# Autodesk Inventor assembly: raspi
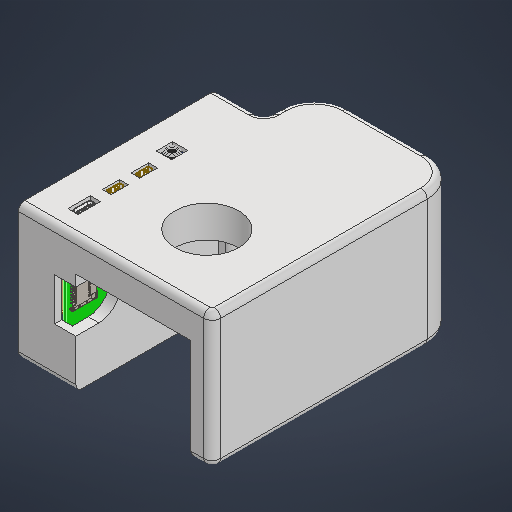
[picture p0: Inventor's stored thumbnail of the model, 512x512]
Saved by Autodesk Inventor 2025.3 (Build 293356030, 356C)
## iProperties
Created: 2025-09-19
Part Number: raspi
Document SubType Name: Assembly
Designer: river
Author: river
## Documents named in this file (4)
- C:\Users\river\OneDrive\Documentos\protesis V2\raspi.iam
- C:\Users\river\OneDrive\Documentos\sync\Part4.ipt
- C:\Users\river\Downloads\self-locking-button-switch-lay37-pbcy-green-1.snapshot.1(1)\Self-locking button switch LAY37 (PBCY) Green\Self-locking button switch LAY37 (PBCY) Green\Self-locking button switch LAY37 .ipt
- C:\Users\river\Downloads\raspberry-pi-4-model-b-1.snapshot.3\Raspberry Pi 4 Model B\Raspberry Pi 4 Model B\Raspberry Pi 4 Model B.ipt
## Components (3 placed, 3 different names)
1. Raspberry Pi 4 Model B:1 — Mate:5, Angle:1
2. Part4:1 — Mate:1, Mate:2, Mate:3, Mate:4, Mate:5, Angle:1
3. Self-locking button switch LAY37 :1 — Mate:2, Mate:3, Mate:4
## Relationships (6: Mate 5, Angle 1)
- Mate:1: Part4:1
- Mate:2: Part4:1 ↔ Self-locking button switch LAY37 :1
- Mate:3: Part4:1 ↔ Self-locking button switch LAY37 :1
- Mate:4: Part4:1 ↔ Self-locking button switch LAY37 :1
- Mate:5 (3 mm): Raspberry Pi 4 Model B:1 ↔ Part4:1
- Angle:1 (0 deg): Raspberry Pi 4 Model B:1 ↔ Part4:1
